# Autodesk Inventor assembly: ElectronicsSideMount_1
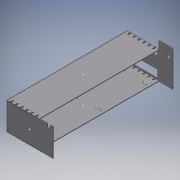
[picture p0: Inventor's stored thumbnail of the model, 180x180]
Saved by Autodesk Inventor 2016 (Build 200138000, 138)
## iProperties
Created: 2017-10-18
Part Number: ElectronicsSideMount_1
Document SubType Name: Assembly
Designer: jcj2131
Author: jcj2131
## Documents named in this file (6)
- C:\Users\jcj2131\Downloads\FinalVersion\ElectronicsSideMount_1.iam
- C:\Users\jcj2131\Downloads\FinalVersion\3DPrinterBracket_bottom_Long_1%2F8.ipt
- C:\Users\jcj2131\Downloads\FinalVersion\3DPrinterBracket_end_long_1%2F8.ipt
- C:\Users\jcj2131\Downloads\FinalVersion\3DPrinterBracket_Top_Long_1%2F8.ipt
- C:\Users\jcj2131\Downloads\FinalVersion\3DprinterSideBracket_2.0_noLCD_1%2F8.ipt
- C:\Users\jcj2131\Downloads\FinalVersion\3DprinterSideBracket_2.0_noLCD_1%2F8_back.ipt
## Components (5 placed, 5 different names)
1. 3DPrinterBracket_bottom_Long_1%2F8:1 — Rigid:5, Rigid:7, Rigid:8
2. 3DPrinterBracket_end_long_1%2F8:1 — Rigid:7
3. 3DPrinterBracket_Top_Long_1%2F8:1 — Rigid:6
4. 3DprinterSideBracket_2.0_noLCD_1%2F8:1 — Rigid:5, Rigid:6
5. 3DprinterSideBracket_2.0_noLCD_1%2F8_back:1 — Rigid:8
## Relationships (4: WeldJoint 4)
- Rigid:5 [WeldJoint]: 3DPrinterBracket_bottom_Long_1%2F8:1 ↔ 3DprinterSideBracket_2.0_noLCD_1%2F8:1
- Rigid:6 [WeldJoint]: 3DPrinterBracket_Top_Long_1%2F8:1 ↔ 3DprinterSideBracket_2.0_noLCD_1%2F8:1
- Rigid:7 [WeldJoint]: 3DPrinterBracket_bottom_Long_1%2F8:1 ↔ 3DPrinterBracket_end_long_1%2F8:1
- Rigid:8 [WeldJoint]: 3DPrinterBracket_bottom_Long_1%2F8:1 ↔ 3DprinterSideBracket_2.0_noLCD_1%2F8_back:1
